# Autodesk Inventor assembly: motor_test_prototype_assembly
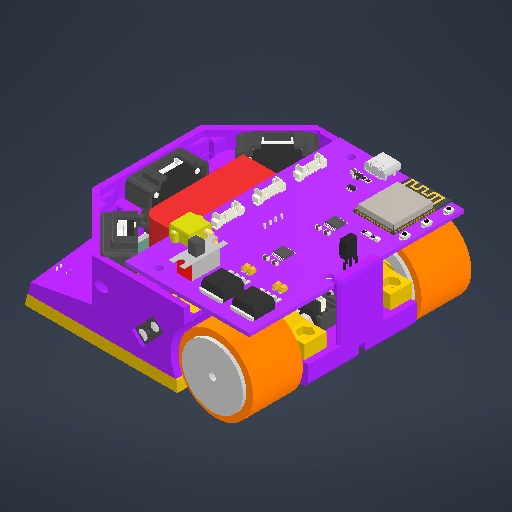
[picture p0: Inventor's stored thumbnail of the model, 512x512]
Saved by Autodesk Inventor 2025 (Build 290162000, 162)
## iProperties
Created: 2024-01-31
Part Number: motor_test_prototype_assembly
Document SubType Name: Assembly
Designer: Simak
Author: Simak
## Documents named in this file (13)
- C:\_desktop\GitHub\Sumec-MiniSumo\-3D-\motor_test_prototype_assembly.iam
- C:\_desktop\GitHub\Sumec-MiniSumo\-3D-\mech._parts\base_plate_v2.ipt
- C:\_desktop\GitHub\Sumec-MiniSumo\-3D-\el._parts\PCBs\QRE MiniBoards\QRE MiniBoards\QRE_MiniBoards_Board.iam
- C:\_desktop\GitHub\Sumec-MiniSumo\-3D-\mech._parts\JSUMO_Wheel_33x25mm.ipt
- C:\_desktop\GitHub\Sumec-MiniSumo\-3D-\el._parts\3s_lipo.ipt
- C:\_desktop\GitHub\Sumec-MiniSumo\-3D-\el._parts\2s_lipo.ipt
- C:\_desktop\GitHub\Sumec-MiniSumo\-3D-\_main_body_parts\TF-Luna_holder\TF-Luna_holder_sestava_v2.iam
- C:\_desktop\GitHub\Sumec-MiniSumo\-3D-\el._parts\SensorSharpDigital\side_senzor.iam
- C:\_desktop\GitHub\Sumec-MiniSumo\-3D-\mech._parts\miniboard_nutt_holder.ipt
- C:\_desktop\GitHub\Sumec-MiniSumo\-3D-\mech._parts\motor_C_clamp.ipt
- C:\_desktop\GitHub\Sumec-MiniSumo\-3D-\el._parts\pololu_12v_650rpm-cb-enc-side-con.ipt
- C:\_desktop\GitHub\Sumec-MiniSumo\-3D-\_main_body_parts\body-motor_test_prototype.ipt
- C:\_desktop\GitHub\Sumec-MiniSumo\-3D-\el._parts\PCBs\main board\sumec.iam
## Components (16 placed, 12 different names)
1. base_plate_v2:1 — Proti sobě:3, Stejný směr:2, Vložit:1, Proti sobě:44, Stejný směr:18, Stejný směr:19
2. QRE_MiniBoards_Board:1 [sub-assembly] — Proti sobě:3, Stejný směr:2, Vložit:1, Proti sobě:30, Stejný směr:17, Vložit:10
3. JSUMO_Wheel_33x25mm:1 — Proti sobě:11, Proti sobě:42
4. JSUMO_Wheel_33x25mm:2 — Proti sobě:11, Proti sobě:43
5. 3s_lipo:1
6. 2s_lipo:1
7. TF-Luna_holder_sestava_v2:1 [sub-assembly]
8. side_senzor:1 [sub-assembly]
9. side_senzor:2 [sub-assembly]
10. miniboard_nutt_holder:1 — Proti sobě:30, Stejný směr:17, Vložit:10
11. motor_C_clamp:1
12. motor_C_clamp:2
13. pololu_12v_650rpm-cb-enc-side-con:1 — Proti sobě:43
14. pololu_12v_650rpm-cb-enc-side-con:2 — Proti sobě:42
15. body-motor_test_prototype:1 — Proti sobě:44, Stejný směr:18, Stejný směr:19, Proti sobě:45, Proti sobě:46, Stejný směr:20
16. sumec:1 [sub-assembly] — Proti sobě:45, Proti sobě:46, Stejný směr:20
## Relationships (15: Mate 8, Flush 5, Insert 2)
- Proti sobě:3 [Mate] (1 mm): base_plate_v2:1 ↔ QRE_MiniBoards_Board:1
- Stejný směr:2 [Flush] (4.75 mm): base_plate_v2:1 ↔ QRE_MiniBoards_Board:1
- Vložit:1 [Insert]: base_plate_v2:1 ↔ QRE_MiniBoards_Board:1
- Proti sobě:11 [Mate]: JSUMO_Wheel_33x25mm:1 ↔ JSUMO_Wheel_33x25mm:2
- Proti sobě:30 [Mate]: QRE_MiniBoards_Board:1 ↔ miniboard_nutt_holder:1
- Stejný směr:17 [Flush]: QRE_MiniBoards_Board:1 ↔ miniboard_nutt_holder:1
- Vložit:10 [Insert]: QRE_MiniBoards_Board:1 ↔ miniboard_nutt_holder:1
- Proti sobě:42 [Mate]: JSUMO_Wheel_33x25mm:1 ↔ pololu_12v_650rpm-cb-enc-side-con:2
- Proti sobě:43 [Mate]: JSUMO_Wheel_33x25mm:2 ↔ pololu_12v_650rpm-cb-enc-side-con:1
- Proti sobě:44 [Mate]: base_plate_v2:1 ↔ body-motor_test_prototype:1
- Stejný směr:18 [Flush]: base_plate_v2:1 ↔ body-motor_test_prototype:1
- Stejný směr:19 [Flush]: base_plate_v2:1 ↔ body-motor_test_prototype:1
- Proti sobě:45 [Mate]: body-motor_test_prototype:1 ↔ sumec:1
- Proti sobě:46 [Mate]: body-motor_test_prototype:1 ↔ sumec:1
- Stejný směr:20 [Flush]: body-motor_test_prototype:1 ↔ sumec:1
## Named parameters: Finish1_Area = 2.15
note: some values were not read from the file. Shown as the stored number, unit unknown: "Finish1_Area".
